# Autodesk Inventor assembly: assembled-feed
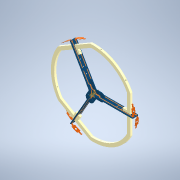
[picture p0: Inventor's stored thumbnail of the model, 180x180]
Saved by Autodesk Inventor 2021 (Build 250183000, 183)
## iProperties
Created: 2020-09-03
Part Number: assembled-feed
Document SubType Name: Assembly
Designer: dsouthall
Author: dsouthall
## iProperties of the stored document tri-slot-hub_with_copper.iam
Created: 2020-11-17
Part Number: tri-slot-hub_with_copper
Description: FreeCAD Model
Document SubType Name: Assembly
Designer: dsouthall
Authority: Unknown
Sending System: FreeCAD
Preprocessor: Open CASCADE STEP processor 7.3
Title: C:/Users/dsouthall/OneDrive - The University of Chicago/Hpol/hpol-prototype/design/Feed Design/tri-slot-hub/tri-slot-hub_with_copper.stp
Author: Author
## iProperties of the stored document board_solid#F.Cu.ipt
Created: 2020-11-17
Part Number: board_solid#F.Cu
Material: Generic
Document SubType Name: Modeling
Designer: dsouthall
Density: 1 g/cm^3
Appearance: Default
Author: dsouthall
## iProperties of the stored document coppers_drilled#F.Cu.ipt
Created: 2020-11-17
Part Number: coppers_drilled#F.Cu
Material: Generic
Document SubType Name: Modeling
Designer: dsouthall
Density: 1 g/cm^3
Appearance: Default
Author: dsouthall
## Documents named in this file (8)
- C:\Users\dsouthall\OneDrive - The University of Chicago\Hpol\hpol-prototype\design\Tri-Slot\Model 8 in\assembled-feed.iam
- C:\Users\dsouthall\OneDrive - The University of Chicago\Hpol\hpol-prototype\design\Tri-Slot\Model 8 in\assembled-feed_feedline_8in.iam
- C:\Users\dsouthall\OneDrive - The University of Chicago\Hpol\hpol-prototype\design\Tri-Slot\Model 8 in\source\insert_8in.ipt
- **C:\Users\dsouthall\OneDrive - The University of Chicago\Hpol\hpol-prototype\design\Tri-Slot\Model 8 in\assembled-feed.iam*LocalDocs*xAaaaauaaAaaaaaaaAaaaanutLe*tri-slot-hub_with_copper.iam
- C:\Users\dsouthall\OneDrive - The University of Chicago\Hpol\hpol-prototype\design\Tri-Slot\Model 8 in\source\hub\COMPOUND.ipt
- C:\Users\dsouthall\OneDrive - The University of Chicago\Hpol\hpol-prototype\design\Feed Design\tri-slot-hub\tri-slot-hub_with_copper.stp
- **C:\Users\dsouthall\OneDrive - The University of Chicago\Hpol\hpol-prototype\design\Tri-Slot\Model 8 in\assembled-feed.iam*LocalDocs*xAaaaauaaAaaaaaaaAaaaagoyTg*board_solid#F.Cu.ipt
- **C:\Users\dsouthall\OneDrive - The University of Chicago\Hpol\hpol-prototype\design\Tri-Slot\Model 8 in\assembled-feed.iam*LocalDocs*xAaaaq5caAaaaaaaaAaaaq2x2Ke*coppers_drilled#F.Cu.ipt
## Components (8 placed, 4 different names)
1. assembled-feed_feedline_8in:1 [sub-assembly] — Insert:4, Insert:6, Flush:2, Flush:3, Mate:5, Angle:4
2. assembled-feed_feedline_8in:2 [sub-assembly] — Insert:1, Insert:5, Mate:3, Mate:4, Flush:2, Mate:10
3. assembled-feed_feedline_8in:3 [sub-assembly] — Insert:2, Insert:3, Flush:3
4. insert_8in:1 — Insert:5, Insert:6, Mate:1, Angle:3
5. insert_8in:2 — Insert:1, Insert:2
6. insert_8in:3 — Insert:3, Insert:4
7. tri-slot-hub_with_copper:1 [sub-assembly] — Insert:7, Angle:2, Mate:3, Mate:4, Mate:5
8. COMPOUND:1 — Insert:7, Angle:2
## Relationships (23: Mate 10, Insert 7, Flush 3, Angle 3)
- Flush:1 (-3.9973 mm)
- Insert:1: assembled-feed_feedline_8in:2 ↔ insert_8in:2
- Insert:2: assembled-feed_feedline_8in:3 ↔ insert_8in:2
- Insert:3: assembled-feed_feedline_8in:3 ↔ insert_8in:3
- Insert:4: assembled-feed_feedline_8in:1 ↔ insert_8in:3
- Insert:5: assembled-feed_feedline_8in:2 ↔ insert_8in:1
- Insert:6: assembled-feed_feedline_8in:1 ↔ insert_8in:1
- Insert:7: tri-slot-hub_with_copper:1 ↔ COMPOUND:1
- Angle:2 (0 deg): tri-slot-hub_with_copper:1 ↔ COMPOUND:1
- Mate:1: insert_8in:1
- Angle:3 (0 deg): insert_8in:1
- Mate:2
- Mate:3: assembled-feed_feedline_8in:2 ↔ tri-slot-hub_with_copper:1
- Mate:4: assembled-feed_feedline_8in:2 ↔ tri-slot-hub_with_copper:1
- Flush:2: assembled-feed_feedline_8in:1 ↔ assembled-feed_feedline_8in:2
- Flush:3: assembled-feed_feedline_8in:1 ↔ assembled-feed_feedline_8in:3
- Mate:5: assembled-feed_feedline_8in:1 ↔ tri-slot-hub_with_copper:1
- Mate:6
- Mate:7
- Mate:9
- Mate:10 (-7 mm): assembled-feed_feedline_8in:2
- Angle:4 (0 deg): assembled-feed_feedline_8in:1
- Mate:11 (-3.9973 mm)
